# Autodesk Inventor assembly: Winch Assembly
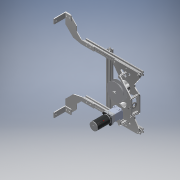
[picture p0: Inventor's stored thumbnail of the model, 180x180]
Saved by Autodesk Inventor 2019.4 (Build 234330000, 330)
## iProperties
Created: 2020-01-24
Part Number: Winch Assembly
Document SubType Name: Assembly
Designer: Mark
Mass: 1680.05 g
Surface Area: 4431.16 cm^2
Volume: 754.263 cm^3
Density: 2.22741 g/cm^3
Author: Mark
## Documents named in this file (15)
- C:\Users\Mark\Desktop\7738 Helion Engineering\7738-2020\Ratchet Winch\Winch Assembly.iam
- C:\Users\Mark\Desktop\7738 Helion Engineering\7738-2020\Ratchet Winch\VersaPlanetary_v2_Two_Stage_100_1_with_BAG.ipt
- C:\Users\Mark\Desktop\7738 Helion Engineering\7738-2020\Ratchet Winch\Right Plate.ipt
- C:\Users\Mark\Desktop\7738 Helion Engineering\7738-2020\Ratchet Winch\0_500_Hex_ID_x_1_125_OD_x_0_313_WD_Flanged_Bearing_v2_217-3875.ipt
- C:\Users\Mark\Desktop\7738 Helion Engineering\7738-2020\Elevator MK2\Pulley.ipt
- C:\Users\Mark\Desktop\7738 Helion Engineering\7738-2020\CAD\Gearbox\F6800.ipt
- C:\Users\Mark\Desktop\7738 Helion Engineering\7738-2020\Ratchet Winch\Left Plate.ipt
- C:\Users\Mark\Desktop\7738 Helion Engineering\7738-2020\Elevator MK2\Smol Hex Shaft.ipt
- C:\Users\Mark\Desktop\7738 Helion Engineering\7738-2020\Ratchet Winch\An Extrusion.ipt
- C:\Users\Mark\Desktop\7738 Helion Engineering\7738-2020\Elevator MK2\Bottom Pneumatic Extrusion.ipt
- C:\Users\Mark\Desktop\7738 Helion Engineering\7738-2020\Elevator MK2\M6 Eye Bolt.ipt
- C:\Users\Mark\Desktop\7738 Helion Engineering\7738-2020\Ratchet Winch\31 mm spacer.ipt
- C:\Users\Mark\Desktop\7738 Helion Engineering\7738-2020\Ratchet Winch\Special 3d printer pulley.ipt
- C:\Users\Mark\Desktop\7738 Helion Engineering\7738-2020\Ratchet Winch\Support Plate.ipt
- C:\Users\Mark\Desktop\7738 Helion Engineering\7738-2020\Ratchet Winch\Small connector.ipt
## Components (23 placed, 14 different names)
1. VersaPlanetary_v2_Two_Stage_100_1_with_BAG:1 — Mate:16, Mate:17, Mate:18
2. Right Plate:1 — Mate:4, Mate:5, Mate:10, Mate:11, Flush:3, Mate:14, Mate:25, Mate:26, Mate:27, Flush:10, Flush:11, Mate:30, Mate:31, Mate:32, Mate:33, Mate:36, Mate:37, Mate:38, Mate:39
3. 0_500_Hex_ID_x_1_125_OD_x_0_313_WD_Flanged_Bearing_v2_217-3875:1 — Mate:4, Mate:5, Mate:6
4. Pulley:1 — Mate:6, Mate:19, Mate:47
5. Pulley:2 — Mate:22, Mate:48
6. F6800:1 — Mate:10, Mate:11, Mate:13
7. F6800:2 — Mate:20, Mate:21, Mate:22
8. Left Plate:1 — Mate:14, Mate:16, Mate:17, Mate:18, Mate:19, Mate:20, Mate:21, Mate:26, Mate:27, Mate:28, Mate:29, Mate:34, Mate:35, Mate:41, Mate:47, Mate:48
9. Smol Hex Shaft:1 — Mate:13, Flush:3, Flush:12, Mate:42
10. An Extrusion:1 — Mate:23, Flush:6, Flush:7, Mate:25, Flush:10, Flush:15, Mate:44
11. An Extrusion:2 — Mate:23, Flush:6, Flush:7, Mate:24, Flush:8, Flush:9, Flush:11, Mate:43, Flush:13, Flush:14
12. Bottom Pneumatic Extrusion:1 — Mate:24, Flush:8, Flush:9
13. M6 Eye Bolt:1 — Mate:28, Mate:29
14. 31 mm spacer:1 — Mate:30, Mate:31
15. 31 mm spacer:2 — Mate:32, Mate:33
16. 31 mm spacer:3 — Mate:34, Mate:35
17. 31 mm spacer:4 — Mate:36, Mate:37
18. 31 mm spacer:5 — Mate:38, Mate:39
19. Special 3d printer pulley:1 — Mate:41, Flush:12, Mate:42
20. Support Plate:1 — Mate:43, Flush:13, Flush:14, Flush:16, Mate:45, Flush:17, Flush:18
21. Support Plate:2 — Flush:15, Mate:44, Flush:16, Flush:19, Flush:20, Mate:46
22. Small connector:1 — Mate:45, Flush:17, Flush:18
23. Small connector:2 — Flush:19, Flush:20, Mate:46
## Relationships (55: Mate 39, Flush 16)
- Mate:4: Right Plate:1 ↔ 0_500_Hex_ID_x_1_125_OD_x_0_313_WD_Flanged_Bearing_v2_217-3875:1
- Mate:5: Right Plate:1 ↔ 0_500_Hex_ID_x_1_125_OD_x_0_313_WD_Flanged_Bearing_v2_217-3875:1
- Mate:6: 0_500_Hex_ID_x_1_125_OD_x_0_313_WD_Flanged_Bearing_v2_217-3875:1 ↔ Pulley:1
- Mate:10: Right Plate:1 ↔ F6800:1
- Mate:11: Right Plate:1 ↔ F6800:1
- Mate:13: F6800:1 ↔ Smol Hex Shaft:1
- Flush:3: Right Plate:1 ↔ Smol Hex Shaft:1
- Mate:14 (31 mm): Right Plate:1 ↔ Left Plate:1
- Mate:16: VersaPlanetary_v2_Two_Stage_100_1_with_BAG:1 ↔ Left Plate:1
- Mate:17: VersaPlanetary_v2_Two_Stage_100_1_with_BAG:1 ↔ Left Plate:1
- Mate:18: VersaPlanetary_v2_Two_Stage_100_1_with_BAG:1 ↔ Left Plate:1
- Mate:19 (0.75 mm): Pulley:1 ↔ Left Plate:1
- Mate:20: F6800:2 ↔ Left Plate:1
- Mate:21: F6800:2 ↔ Left Plate:1
- Mate:22: Pulley:2 ↔ F6800:2
- Mate:23 (239 mm): An Extrusion:1 ↔ An Extrusion:2
- Flush:6: An Extrusion:1 ↔ An Extrusion:2
- Flush:7: An Extrusion:1 ↔ An Extrusion:2
- Mate:24: An Extrusion:2 ↔ Bottom Pneumatic Extrusion:1
- Flush:8 (100 mm): An Extrusion:2 ↔ Bottom Pneumatic Extrusion:1
- Flush:9: An Extrusion:2 ↔ Bottom Pneumatic Extrusion:1
- Mate:25: Right Plate:1 ↔ An Extrusion:1
- Mate:26: Right Plate:1 ↔ Left Plate:1
- Mate:27: Right Plate:1 ↔ Left Plate:1
- Flush:10: Right Plate:1 ↔ An Extrusion:1
- Flush:11: Right Plate:1 ↔ An Extrusion:2
- Mate:28: Left Plate:1 ↔ M6 Eye Bolt:1
- Mate:29: Left Plate:1 ↔ M6 Eye Bolt:1
- Mate:30: Right Plate:1 ↔ 31 mm spacer:1
- Mate:31: Right Plate:1 ↔ 31 mm spacer:1
- Mate:32: Right Plate:1 ↔ 31 mm spacer:2
- Mate:33: Right Plate:1 ↔ 31 mm spacer:2
- Mate:34: Left Plate:1 ↔ 31 mm spacer:3
- Mate:35: Left Plate:1 ↔ 31 mm spacer:3
- Mate:36: Right Plate:1 ↔ 31 mm spacer:4
- Mate:37: Right Plate:1 ↔ 31 mm spacer:4
- Mate:38: Right Plate:1 ↔ 31 mm spacer:5
- Mate:39: Right Plate:1 ↔ 31 mm spacer:5
- Mate:41 (1 mm): Left Plate:1 ↔ Special 3d printer pulley:1
- Flush:12: Smol Hex Shaft:1 ↔ Special 3d printer pulley:1
- Mate:42: Smol Hex Shaft:1 ↔ Special 3d printer pulley:1
- Mate:43: An Extrusion:2 ↔ Support Plate:1
- Flush:13: An Extrusion:2 ↔ Support Plate:1
- Flush:14 (-90 mm): An Extrusion:2 ↔ Support Plate:1
- Flush:15: An Extrusion:1 ↔ Support Plate:2
- Mate:44: An Extrusion:1 ↔ Support Plate:2
- Flush:16: Support Plate:1 ↔ Support Plate:2
- Mate:45: Support Plate:1 ↔ Small connector:1
- Flush:17: Support Plate:1 ↔ Small connector:1
- Flush:18: Support Plate:1 ↔ Small connector:1
- Flush:19: Support Plate:2 ↔ Small connector:2
- Flush:20: Support Plate:2 ↔ Small connector:2
- Mate:46: Support Plate:2 ↔ Small connector:2
- Mate:47 (2.5 mm): Pulley:1 ↔ Left Plate:1
- Mate:48 (2.5 mm): Pulley:2 ↔ Left Plate:1
